# Autodesk Inventor assembly: Assembly_cube_StormChip_v4
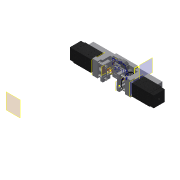
[picture p0: Inventor's stored thumbnail of the model, 180x180]
Saved by Autodesk Inventor 2019 (Build 230136000, 136)
## iProperties
Created: 2018-06-27
Part Number: Assembly_cube_StormChip_v4
Material: Generisch
Document SubType Name: Assembly
Designer: diederichbenedict
Author: diederichbenedict
## Documents named in this file (14)
- C:\Users\diederichbenedict\Dropbox\Dokumente\Promotion\PROJECTS\STORMoChip\INVENTOR\10_Cube_Base\Assembly_cube_StormChip_v5.iam
- C:\Users\diederichbenedict\Dropbox\Dokumente\Promotion\PROJECTS\STORMoChip\INVENTOR\10_Cube_Base\10_Cube_3x_v0.ipt
- C:\Users\diederichbenedict\Dropbox\Dokumente\Promotion\PROJECTS\STORMoChip\INVENTOR\10_Cube_Base\10_Lid_el_3x_v0.ipt
- C:\Users\diederichbenedict\Dropbox\Dokumente\Promotion\PROJECTS\STORMoChip\INVENTOR\10_Cube_Base\LASER_640nm.ipt
- C:\Users\diederichbenedict\Dropbox\Dokumente\Promotion\PROJECTS\STORMoChip\INVENTOR\10_Cube_Base\40_XYZ_Adapter_Flattener.ipt
- C:\Users\diederichbenedict\Dropbox\Dokumente\Promotion\PROJECTS\STORMoChip\INVENTOR\10_Cube_Base\00_dSTORM_Chip.ipt
- C:\Users\diederichbenedict\Dropbox\Dokumente\Promotion\PROJECTS\STORMoChip\INVENTOR\10_Cube_Base\Raman2Go_ProbenhalterXY-Verstellung_mit_Adapterplatten.iam
- C:\Users\diederichbenedict\Dropbox\Dokumente\Promotion\PROJECTS\STORMoChip\INVENTOR\10_Cube_Base\20_Adapter_Laser_Thorlabs.ipt
- C:\Users\diederichbenedict\Dropbox\Dokumente\Promotion\PROJECTS\STORMoChip\INVENTOR\10_Cube_Base\00_40mm_Rod_Thorlabs.ipt
- C:\Users\diederichbenedict\Dropbox\Dokumente\Promotion\PROJECTS\STORMoChip\INVENTOR\10_Cube_Base\Assembly_Lens_Thorlabs_Mount_KES400_Bluraylasermount.iam
- C:\Users\diederichbenedict\Dropbox\Dokumente\Promotion\PROJECTS\STORMoChip\INVENTOR\10_Cube_Base\00_KES400_Bluray_Lens.ipt
- C:\Users\diederichbenedict\Dropbox\Dokumente\Promotion\PROJECTS\STORMoChip\INVENTOR\00_Laser_coupling.ipt
- C:\Users\diederichbenedict\Dropbox\Dokumente\Promotion\PROJECTS\STORMoChip\INVENTOR\10_Cube_Base\20_Base_STORMchip_doublesided.ipt
- C:\Users\diederichbenedict\Dropbox\Dokumente\Promotion\PROJECTS\STORMoChip\INVENTOR\10_Cube_Base\20_Adapter_Bluray_KES400_Lens_Thorlabs.ipt
## Components (20 placed, 13 different names)
1. 10_Cube_3x_v0:1 — Einfügen:1, Einfügen:2, Passend:1, Winkel:2, Winkel:3
2. 10_Lid_el_3x_v0:1 — Einfügen:1, Einfügen:2
3. 40_XYZ_Adapter_Flattener:1
4. 00_dSTORM_Chip:1 — Passend:1, Winkel:3
5. 00_dSTORM_Chip:2 — Winkel:2, Mate:20
6. 20_Base_STORMchip_doublesided:1 — Angle:10, Mate:14, Mate:15, Mate:16, Angle:11, Flush:19, Insert:3, Insert:4, Angle:19, Flush:20, Insert:5, Insert:6, Angle:20
7. Raman2Go_ProbenhalterXY-Verstellung_mit_Adapterplatten:2 [sub-assembly] — Angle:10, Mate:14, Mate:15, Mate:20
8. LASER_640nm:3 — Mate:16, Angle:11, Flush:12, Mate:34, Flush:19
9. 20_Adapter_Laser_Thorlabs:1 — Flush:12
10. LASER_640nm:4 — Mate:34, Mate:42, Angle:18, Flush:20, Mate:49
11. 00_Laser_coupling:1 — Mate:48, Mate:49, Mate:52
12. Assembly_Lens_Thorlabs_Mount_KES400_Bluraylasermount:2 [sub-assembly] — Mate:42, Angle:18
13. 00_40mm_Rod_Thorlabs:2 — Insert:3
14. 00_40mm_Rod_Thorlabs:3 — Insert:4, Mate:43
15. 20_Adapter_Bluray_KES400_Lens_Thorlabs:1 — Mate:43, Angle:19, Mate:50, Mate:51, Angle:23
16. 00_40mm_Rod_Thorlabs:4 — Insert:6, Mate:46
17. 00_40mm_Rod_Thorlabs:5 — Insert:5
18. 20_Adapter_Bluray_KES400_Lens_Thorlabs:2 — Mate:46, Angle:20, Mate:47, Angle:21, Angle:22, Mate:50
19. 00_KES400_Bluray_Lens:2 — Mate:51, Mate:52, Angle:23
20. 00_KES400_Bluray_Lens:3 — Mate:47, Mate:48, Angle:21, Angle:22
## Relationships (34: Mate 15, Angle 10, Insert 6, Flush 3)
- Einfügen:1 [Insert]: 10_Cube_3x_v0:1 ↔ 10_Lid_el_3x_v0:1
- Einfügen:2 [Insert]: 10_Cube_3x_v0:1 ↔ 10_Lid_el_3x_v0:1
- Passend:1 [Mate]: 10_Cube_3x_v0:1 ↔ 00_dSTORM_Chip:1
- Winkel:2 [Angle] (0 deg): 10_Cube_3x_v0:1 ↔ 00_dSTORM_Chip:2
- Winkel:3 [Angle] (0 deg): 10_Cube_3x_v0:1 ↔ 00_dSTORM_Chip:1
- Angle:10 (180 deg): 20_Base_STORMchip_doublesided:1 ↔ Raman2Go_ProbenhalterXY-Verstellung_mit_Adapterplatten:2
- Mate:14: 20_Base_STORMchip_doublesided:1 ↔ Raman2Go_ProbenhalterXY-Verstellung_mit_Adapterplatten:2
- Mate:15: 20_Base_STORMchip_doublesided:1 ↔ Raman2Go_ProbenhalterXY-Verstellung_mit_Adapterplatten:2
- Mate:16: 20_Base_STORMchip_doublesided:1 ↔ LASER_640nm:3
- Angle:11 (0 deg): 20_Base_STORMchip_doublesided:1 ↔ LASER_640nm:3
- Flush:12: LASER_640nm:3 ↔ 20_Adapter_Laser_Thorlabs:1
- Mate:20: 00_dSTORM_Chip:2 ↔ Raman2Go_ProbenhalterXY-Verstellung_mit_Adapterplatten:2
- Mate:34: LASER_640nm:3 ↔ LASER_640nm:4
- Mate:42 (30 mm): LASER_640nm:4 ↔ Assembly_Lens_Thorlabs_Mount_KES400_Bluraylasermount:2
- Angle:18 (0 deg): LASER_640nm:4 ↔ Assembly_Lens_Thorlabs_Mount_KES400_Bluraylasermount:2
- Flush:19 (4 mm): 20_Base_STORMchip_doublesided:1 ↔ LASER_640nm:3
- Insert:3: 20_Base_STORMchip_doublesided:1 ↔ 00_40mm_Rod_Thorlabs:2
- Insert:4: 20_Base_STORMchip_doublesided:1 ↔ 00_40mm_Rod_Thorlabs:3
- Mate:43: 00_40mm_Rod_Thorlabs:3 ↔ 20_Adapter_Bluray_KES400_Lens_Thorlabs:1
- Angle:19 (0 deg): 20_Base_STORMchip_doublesided:1 ↔ 20_Adapter_Bluray_KES400_Lens_Thorlabs:1
- Flush:20 (4 mm): 20_Base_STORMchip_doublesided:1 ↔ LASER_640nm:4
- Insert:5: 20_Base_STORMchip_doublesided:1 ↔ 00_40mm_Rod_Thorlabs:5
- Insert:6: 20_Base_STORMchip_doublesided:1 ↔ 00_40mm_Rod_Thorlabs:4
- Mate:46: 00_40mm_Rod_Thorlabs:4 ↔ 20_Adapter_Bluray_KES400_Lens_Thorlabs:2
- Angle:20 (0 deg): 20_Base_STORMchip_doublesided:1 ↔ 20_Adapter_Bluray_KES400_Lens_Thorlabs:2
- Mate:47: 20_Adapter_Bluray_KES400_Lens_Thorlabs:2 ↔ 00_KES400_Bluray_Lens:3
- Mate:48: 00_Laser_coupling:1 ↔ 00_KES400_Bluray_Lens:3
- Mate:49: LASER_640nm:4 ↔ 00_Laser_coupling:1
- Angle:21 (0 deg): 20_Adapter_Bluray_KES400_Lens_Thorlabs:2 ↔ 00_KES400_Bluray_Lens:3
- Angle:22 (0 deg): 20_Adapter_Bluray_KES400_Lens_Thorlabs:2 ↔ 00_KES400_Bluray_Lens:3
- Mate:50 (38 mm): 20_Adapter_Bluray_KES400_Lens_Thorlabs:1 ↔ 20_Adapter_Bluray_KES400_Lens_Thorlabs:2
- Mate:51: 20_Adapter_Bluray_KES400_Lens_Thorlabs:1 ↔ 00_KES400_Bluray_Lens:2
- Mate:52: 00_Laser_coupling:1 ↔ 00_KES400_Bluray_Lens:2
- Angle:23 (0 deg): 20_Adapter_Bluray_KES400_Lens_Thorlabs:1 ↔ 00_KES400_Bluray_Lens:2
